# Autodesk Inventor assembly: Assembly_Post_v0
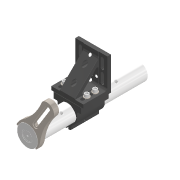
[picture p0: Inventor's stored thumbnail of the model, 180x180]
Saved by Autodesk Inventor 2022 (Build 260153000, 153)
## iProperties
Created: 2022-04-28
Part Number: Assembly_Post_v0
Document SubType Name: Assembly
Designer: diederichbenedict
Author: diederichbenedict
## Documents named in this file (5)
- E:\GitHub\SIMMO\INVENTOR\Assembly_Post_v0.iam
- E:\GitHub\SIMMO\INVENTOR\00_C1515_M-Step.ipt
- E:\GitHub\SIMMO\INVENTOR\00_PF175B-Step.ipt
- E:\GitHub\SIMMO\INVENTOR\00_P125_M-Step.ipt
- E:\GitHub\SIMMO\INVENTOR\00_PB4_M-Step.ipt
## Components (5 placed, 4 different names)
1. 00_PF175B-Step:1
2. 00_PB4_M-Step:1
3. 00_P125_M-Step:1
4. 00_C1515_M-Step:1
5. 00_P125_M-Step:2
## Relationships (4: Insert 3, Mate 1)
- [Insert]: 00_P125_M-Step:1 ↔ 00_P125_M-Step:2
- [Mate]: 00_C1515_M-Step:1 ↔ 00_P125_M-Step:2
- [Insert]: 00_PB4_M-Step:1 ↔ 00_P125_M-Step:1
- [Insert]: 00_PF175B-Step:1 ↔ 00_PB4_M-Step:1
